# Autodesk Inventor assembly: Turret Shooter Assembly
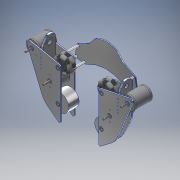
[picture p0: Inventor's stored thumbnail of the model, 180x180]
Saved by Autodesk Inventor 2019.4 (Build 234330000, 330)
## iProperties
Created: 2020-01-06
Part Number: Turret Shooter Assembly
Document SubType Name: Assembly
Designer: admin
Mass: 4067.01 g
Surface Area: 6466.54 cm^2
Volume: 4994.12 cm^3
Density: 0.814359 g/cm^3
Author: admin
## Documents named in this file (14)
- C:\Users\admin\Desktop\FRC 2020 Engineering\GitHub\7738-2020\Turret\Turret Shooter Assembly.iam
- C:\Users\admin\Desktop\FRC 2020 Engineering\GitHub\7738-2020\Turret\Omni Wheel\3_25_Omni-Directional_Wheel_217-4775.iam
- C:\Users\admin\Desktop\FRC 2020 Engineering\GitHub\7738-2020\Power Cell.ipt
- C:\Users\admin\Desktop\FRC 2020 Engineering\GitHub\7738-2020\Turret\Flywheel.ipt
- C:\Users\admin\Desktop\FRC 2020 Engineering\GitHub\7738-2020\Turret\Mini CIM\Mini_CIM_Motor_217-3371.ipt
- C:\Users\admin\Desktop\FRC 2020 Engineering\GitHub\7738-2020\CAD\Gearbox\F6800.ipt
- C:\Users\admin\Desktop\FRC 2020 Engineering\GitHub\7738-2020\Turret\Flywheel Bracket 1.ipt
- C:\Users\admin\Desktop\FRC 2020 Engineering\GitHub\7738-2020\Turret\Flywheel Bracket 2.ipt
- C:\Users\admin\Desktop\FRC 2020 Engineering\GitHub\7738-2020\Turret\Pivot Plate.ipt
- C:\Users\admin\Desktop\FRC 2020 Engineering\GitHub\7738-2020\Turret\Slewing Bearing.ipt
- C:\Users\admin\Desktop\FRC 2020 Engineering\GitHub\7738-2020\CAD\Gearbox\F6804.ipt
- C:\Users\admin\Desktop\FRC 2020 Engineering\GitHub\7738-2020\Turret\Pivot Plate Idle.ipt
- C:\Users\admin\Desktop\FRC 2020 Engineering\GitHub\7738-2020\Turret\Ball Stop.ipt
- C:\Users\admin\Desktop\FRC 2020 Engineering\GitHub\7738-2020\Turret\Stopper Spacers.ipt
## Components (32 placed, 13 different names)
1. 3_25_Omni-Directional_Wheel_217-4775:1 [sub-assembly] — Angle:1, Mate:17, Flush:7, Flush:8, Mate:100, Mate:101
2. Power Cell:1 — Mate:5, Mate:6
3. Flywheel:1 — Flush:3, Mate:3, Flush:6, Mate:8, Flush:7, Mate:20, Mate:24, Mate:99
4. Mini_CIM_Motor_217-3371:1 — Flush:3, Mate:9, Mate:10
5. F6800:2 — Mate:11, Mate:12
6. Flywheel Bracket 1:1 — Mate:8, Mate:9, Mate:10, Mate:11, Mate:12, Mate:25, Mate:27, Mate:29, Mate:30, Angle:3, Flush:11, Mate:107, Mate:108
7. Flywheel Bracket 2:1 — Mate:20, Mate:22, Mate:23, Mate:28, Angle:2, Mate:70, Mate:74, Mate:75, Mate:76, Mate:103
8. F6800:3 — Mate:22, Mate:23, Mate:24
9. F6800:4 — Mate:28, Mate:32, Mate:104
10. F6800:5 — Mate:25, Mate:27, Mate:101
11. Pivot Plate:1 — Mate:29, Mate:30, Flush:10, Flush:12, Mate:103
12. Slewing Bearing:1
13. F6804:2 — Mate:65, Mate:66
14. 3_25_Omni-Directional_Wheel_217-4775:2 [sub-assembly] — Mate:57, Flush:8, Mate:59, Mate:83, Mate:100
15. Flywheel:2 — Mate:45, Mate:46, Mate:60, Mate:62, Mate:99
16. F6800:6 — Mate:46, Mate:62, Mate:84, Mate:89
17. F6800:7 — Mate:83, Mate:96, Mate:105
18. F6800:8 — Mate:57, Mate:59, Mate:85, Mate:106
19. F6800:9 — Mate:45, Mate:60, Mate:95
20. Pivot Plate Idle:1 — Mate:65, Mate:66, Flush:10, Mate:91, Flush:12, Mate:97, Mate:98
21. Ball Stop:1 — Mate:70, Mate:77, Mate:78, Mate:79, Mate:80, Mate:81, Mate:82, Mate:111, Mate:112, Mate:113
22. Stopper Spacers:1 — Mate:77, Mate:111
23. Stopper Spacers:2 — Mate:78, Mate:113
24. Stopper Spacers:3 — Mate:79, Mate:112
25. Stopper Spacers:4 — Mate:76, Mate:82
26. Stopper Spacers:5 — Mate:75, Mate:80
27. Stopper Spacers:6 — Mate:74, Mate:81
28. Flywheel Bracket 1:2 — Mate:84, Mate:85, Angle:3, Mate:89, Flush:11, Mate:91, Mate:94, Mate:98, Mate:106, Mate:109, Mate:110
29. Flywheel Bracket 2:2 — Mate:95, Mate:96, Mate:97, Mate:102, Mate:104, Mate:105
30. Mini_CIM_Motor_217-3371:2 — Mate:94, Mate:102
31. Mini_CIM_Motor_217-3371:3 — Mate:107, Mate:108
32. Mini_CIM_Motor_217-3371:4 — Mate:109, Mate:110
## Relationships (73: Mate 62, Flush 8, Angle 3)
- Flush:3 (-5 mm): Flywheel:1 ↔ Mini_CIM_Motor_217-3371:1
- Mate:3 (103.5 mm): Flywheel:1
- Mate:5: Power Cell:1
- Mate:6: Power Cell:1
- Flush:5 (103.5 mm)
- Flush:6 (-25 mm): Flywheel:1
- Mate:8: Flywheel:1 ↔ Flywheel Bracket 1:1
- Mate:9: Mini_CIM_Motor_217-3371:1 ↔ Flywheel Bracket 1:1
- Mate:10: Mini_CIM_Motor_217-3371:1 ↔ Flywheel Bracket 1:1
- Mate:11: F6800:2 ↔ Flywheel Bracket 1:1
- Mate:12 (0.2 mm): F6800:2 ↔ Flywheel Bracket 1:1
- Angle:1 (0 deg): 3_25_Omni-Directional_Wheel_217-4775:1
- Mate:17: 3_25_Omni-Directional_Wheel_217-4775:1
- Flush:7 (5.95 mm): 3_25_Omni-Directional_Wheel_217-4775:1 ↔ Flywheel:1
- Mate:20: Flywheel:1 ↔ Flywheel Bracket 2:1
- Mate:22: Flywheel Bracket 2:1 ↔ F6800:3
- Mate:23 (0.2 mm): Flywheel Bracket 2:1 ↔ F6800:3
- Mate:24 (5 mm): Flywheel:1 ↔ F6800:3
- Mate:25: Flywheel Bracket 1:1 ↔ F6800:5
- Mate:27 (0.2 mm): Flywheel Bracket 1:1 ↔ F6800:5
- Mate:28 (0.2 mm): Flywheel Bracket 2:1 ↔ F6800:4
- Mate:29 (0.1 mm): Flywheel Bracket 1:1 ↔ Pivot Plate:1
- Mate:30: Flywheel Bracket 1:1 ↔ Pivot Plate:1
- Mate:32: F6800:4
- Angle:2 (180 deg): Flywheel Bracket 2:1
- Mate:45 (5 mm): Flywheel:2 ↔ F6800:9
- Mate:46 (5 mm): Flywheel:2 ↔ F6800:6
- Mate:57: 3_25_Omni-Directional_Wheel_217-4775:2 ↔ F6800:8
- Flush:8: 3_25_Omni-Directional_Wheel_217-4775:1 ↔ 3_25_Omni-Directional_Wheel_217-4775:2
- Mate:59: 3_25_Omni-Directional_Wheel_217-4775:2 ↔ F6800:8
- Mate:60: Flywheel:2 ↔ F6800:9
- Mate:62: Flywheel:2 ↔ F6800:6
- Mate:65: F6804:2 ↔ Pivot Plate Idle:1
- Mate:66 (0.2 mm): F6804:2 ↔ Pivot Plate Idle:1
- Flush:10: Pivot Plate:1 ↔ Pivot Plate Idle:1
- Mate:70 (55 mm): Flywheel Bracket 2:1 ↔ Ball Stop:1
- Mate:74: Flywheel Bracket 2:1 ↔ Stopper Spacers:6
- Mate:75: Flywheel Bracket 2:1 ↔ Stopper Spacers:5
- Mate:76: Flywheel Bracket 2:1 ↔ Stopper Spacers:4
- Mate:77: Ball Stop:1 ↔ Stopper Spacers:1
- Mate:78: Ball Stop:1 ↔ Stopper Spacers:2
- Mate:79: Ball Stop:1 ↔ Stopper Spacers:3
- Mate:80: Ball Stop:1 ↔ Stopper Spacers:5
- Mate:81: Ball Stop:1 ↔ Stopper Spacers:6
- Mate:82: Ball Stop:1 ↔ Stopper Spacers:4
- Mate:83: 3_25_Omni-Directional_Wheel_217-4775:2 ↔ F6800:7
- Mate:84: F6800:6 ↔ Flywheel Bracket 1:2
- Mate:85: F6800:8 ↔ Flywheel Bracket 1:2
- Angle:3 (180 deg): Flywheel Bracket 1:1 ↔ Flywheel Bracket 1:2
- Mate:89 (0.2 mm): F6800:6 ↔ Flywheel Bracket 1:2
- Flush:11: Flywheel Bracket 1:1 ↔ Flywheel Bracket 1:2
- Mate:91: Pivot Plate Idle:1 ↔ Flywheel Bracket 1:2
- Flush:12: Pivot Plate:1 ↔ Pivot Plate Idle:1
- Mate:94: Flywheel Bracket 1:2 ↔ Mini_CIM_Motor_217-3371:2
- Mate:95: F6800:9 ↔ Flywheel Bracket 2:2
- Mate:96: F6800:7 ↔ Flywheel Bracket 2:2
- Mate:97 (0.1 mm): Pivot Plate Idle:1 ↔ Flywheel Bracket 2:2
- Mate:98 (0.1 mm): Pivot Plate Idle:1 ↔ Flywheel Bracket 1:2
- Mate:99 (209.55 mm): Flywheel:1 ↔ Flywheel:2
- Mate:100 (209.55 mm): 3_25_Omni-Directional_Wheel_217-4775:1 ↔ 3_25_Omni-Directional_Wheel_217-4775:2
- Mate:101: 3_25_Omni-Directional_Wheel_217-4775:1 ↔ F6800:5
- Mate:102: Flywheel Bracket 2:2 ↔ Mini_CIM_Motor_217-3371:2
- Mate:103: Flywheel Bracket 2:1 ↔ Pivot Plate:1
- Mate:104 (209.55 mm): F6800:4 ↔ Flywheel Bracket 2:2
- Mate:105 (0.2 mm): F6800:7 ↔ Flywheel Bracket 2:2
- Mate:106 (0.2 mm): F6800:8 ↔ Flywheel Bracket 1:2
- Mate:107: Flywheel Bracket 1:1 ↔ Mini_CIM_Motor_217-3371:3
- Mate:108: Flywheel Bracket 1:1 ↔ Mini_CIM_Motor_217-3371:3
- Mate:109: Flywheel Bracket 1:2 ↔ Mini_CIM_Motor_217-3371:4
- Mate:110: Flywheel Bracket 1:2 ↔ Mini_CIM_Motor_217-3371:4
- Mate:111: Ball Stop:1 ↔ Stopper Spacers:1
- Mate:112: Ball Stop:1 ↔ Stopper Spacers:3
- Mate:113: Ball Stop:1 ↔ Stopper Spacers:2
